# Autodesk Inventor assembly: Shifting Cylinder Mechanism for Ball Shifter
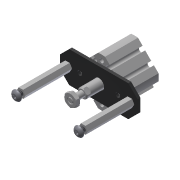
[picture p0: Inventor's stored thumbnail of the model, 180x180]
Saved by Autodesk Inventor 2013 (Build 170138000, 138)
## iProperties
Created: 2013-04-08
Part Number: Shifting Cylinder Mechanism for Ball Shifter
Document SubType Name: Assembly
Designer: Niemitalo_Dan
Author: Niemitalo_Dan
## Documents named in this file (6)
- H:\Nemo\Documents\Robotics\COTS Parts\Ballshifter\Shifting Cylinder Mechanism for Ball Shifter.iam
- H:\Nemo\Documents\Robotics\COTS Parts\Fasteners\Hex Standoff 8-32 x1500.ipt
- H:\Nemo\Documents\Robotics\COTS Parts\Fasteners\8-32 BHCS x375.ipt
- H:\Nemo\Documents\Robotics\COTS Parts\Ballshifter\BS cylinder mounting plate.ipt
- H:\Nemo\Documents\Robotics\COTS Parts\Ballshifter\Ballshifter Cylinder.iam
- H:\Nemo\Documents\Robotics\COTS Parts\Ballshifter\Jam Nut for Ballshifter Cylinder.ipt
## Components (9 placed, 5 different names)
1. Hex Standoff 8-32 x1500:1 — Insert:6
2. Hex Standoff 8-32 x1500:2 — Insert:5, Mate:3
3. 8-32 BHCS x375:1 — Insert:6
4. 8-32 BHCS x375:2 — Insert:5
5. BS cylinder mounting plate:1 — Mate:3
6. 8-32 BHCS x375:3
7. 8-32 BHCS x375:4
8. Ballshifter Cylinder:1 [sub-assembly] — Mate:2, Flush:1
9. Jam Nut for Ballshifter Cylinder:1 — Mate:2, Flush:1
## Relationships (11: Insert 6, Mate 3, Angle 1, Flush 1)
- [Insert]: Hex Standoff 8-32 x1500:1 ↔ BS cylinder mounting plate:1
- [Mate]: Hex Standoff 8-32 x1500:2 ↔ BS cylinder mounting plate:1
- [Insert]: BS cylinder mounting plate:1 ↔ 8-32 BHCS x375:3
- [Insert]: BS cylinder mounting plate:1 ↔ 8-32 BHCS x375:4
- [Insert]: BS cylinder mounting plate:1 ↔ Ballshifter Cylinder:1
- [Angle] (45 deg): BS cylinder mounting plate:1 ↔ Ballshifter Cylinder:1
- Mate:2: Ballshifter Cylinder:1 ↔ Jam Nut for Ballshifter Cylinder:1
- Insert:5 (3.175 mm): Hex Standoff 8-32 x1500:2 ↔ 8-32 BHCS x375:2
- Insert:6 (3.175 mm): Hex Standoff 8-32 x1500:1 ↔ 8-32 BHCS x375:1
- Mate:3: Hex Standoff 8-32 x1500:2 ↔ BS cylinder mounting plate:1
- Flush:1: Ballshifter Cylinder:1 ↔ Jam Nut for Ballshifter Cylinder:1
